# Autodesk Inventor assembly: four-square-11
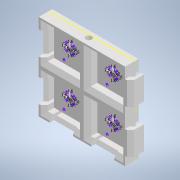
[picture p0: Inventor's stored thumbnail of the model, 180x180]
Saved by Autodesk Inventor 2021 (Build 250183000, 183)
## iProperties
Created: 2020-12-08
Part Number: four-square-11
Document SubType Name: Assembly
Designer: Luke Kamols
Author: Luke Kamols
## Documents named in this file (5)
- C:\Users\Luke Kamols\OneDrive\Documents\Other\Chess\four-square-11.iam
- C:\Users\Luke Kamols\OneDrive\Documents\Other\Chess\one-square.ipt
- C:\Users\Luke Kamols\OneDrive\Documents\Other\Chess\no-join.ipt
- C:\Users\Luke Kamols\OneDrive\Documents\Other\Chess\outside-join.ipt
- C:\Users\Luke Kamols\OneDrive\Documents\Other\Chess\inside-join.ipt
## Components (12 placed, 4 different names)
1. one-square:1 — Mate:1, Flush:1, Flush:2, Mate:2, Flush:3, Flush:4, Mate:12, Mate:13, Flush:14, Mate:14, Mate:15, Flush:15
2. one-square:2 — Mate:1, Flush:1, Flush:2, Flush:5, Mate:3, Mate:8, Mate:9, Flush:12, Flush:16, Mate:16, Mate:17
3. one-square:3 — Mate:2, Flush:3, Flush:4, Mate:4, Mate:5, Flush:7, Mate:10, Flush:13, Mate:11
4. one-square:4 — Flush:5, Mate:3, Mate:4, Flush:6, Flush:8, Flush:9, Mate:6, Mate:7, Flush:10
5. no-join:1 — Mate:5, Flush:6, Flush:7
6. no-join:2 — Flush:8, Flush:9, Mate:6
7. outside-join:1 — Mate:7, Flush:10, Mate:8, Flush:11
8. outside-join:2 — Mate:9, Flush:11, Flush:12
9. inside-join:1 — Mate:10, Flush:13, Mate:11
10. inside-join:2 — Mate:12, Mate:13, Flush:14
11. inside-join:3 — Flush:16, Mate:16, Mate:17
12. inside-join:4 — Mate:14, Mate:15, Flush:15
## Relationships (33: Mate 17, Flush 16)
- Mate:1: one-square:1 ↔ one-square:2
- Flush:1: one-square:1 ↔ one-square:2
- Flush:2: one-square:1 ↔ one-square:2
- Mate:2: one-square:1 ↔ one-square:3
- Flush:3: one-square:1 ↔ one-square:3
- Flush:4: one-square:1 ↔ one-square:3
- Flush:5: one-square:2 ↔ one-square:4
- Mate:3: one-square:2 ↔ one-square:4
- Mate:4: one-square:3 ↔ one-square:4
- Mate:5: one-square:3 ↔ no-join:1
- Flush:6: one-square:4 ↔ no-join:1
- Flush:7: one-square:3 ↔ no-join:1
- Flush:8: one-square:4 ↔ no-join:2
- Flush:9: one-square:4 ↔ no-join:2
- Mate:6: one-square:4 ↔ no-join:2
- Mate:7: one-square:4 ↔ outside-join:1
- Flush:10: one-square:4 ↔ outside-join:1
- Mate:8: one-square:2 ↔ outside-join:1
- Mate:9: one-square:2 ↔ outside-join:2
- Flush:11: outside-join:1 ↔ outside-join:2
- Flush:12: one-square:2 ↔ outside-join:2
- Mate:10 (3 mm): one-square:3 ↔ inside-join:1
- Flush:13: one-square:3 ↔ inside-join:1
- Mate:11: one-square:3 ↔ inside-join:1
- Mate:12 (3 mm): one-square:1 ↔ inside-join:2
- Mate:13: one-square:1 ↔ inside-join:2
- Flush:14: one-square:1 ↔ inside-join:2
- Mate:14 (3 mm): one-square:1 ↔ inside-join:4
- Mate:15: one-square:1 ↔ inside-join:4
- Flush:15: one-square:1 ↔ inside-join:4
- Flush:16: one-square:2 ↔ inside-join:3
- Mate:16 (3 mm): one-square:2 ↔ inside-join:3
- Mate:17: one-square:2 ↔ inside-join:3
